# Autodesk Inventor assembly: Drive Base Assembly
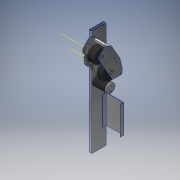
[picture p0: Inventor's stored thumbnail of the model, 180x180]
Saved by Autodesk Inventor 2019.4 (Build 234330000, 330)
## iProperties
Created: 2019-11-02
Part Number: Drive Base Assembly
Document SubType Name: Assembly
Designer: admin
Author: admin
## Documents named in this file (13)
- C:\Users\admin\Desktop\FRC 2020 Engineering\GitHub\7738-CAD-prep\Butterfly Drive Mk2\Butterfly Base\Drive Base Assembly.iam
- C:\Users\admin\Desktop\FRC 2020 Engineering\GitHub\7738-CAD-prep\Butterfly Drive Mk2\Butterfly Base\Main Axle.ipt
- C:\Users\admin\Desktop\FRC 2020 Engineering\GitHub\7738-CAD-prep\Butterfly Drive Mk2\Butterfly Module\Butterfly Drive Module.iam
- C:\Users\admin\Desktop\FRC 2020 Engineering\GitHub\7738-CAD-prep\Butterfly Drive Mk2\Butterfly Base\Side Extrusion.ipt
- C:\Users\admin\Desktop\FRC 2020 Engineering\GitHub\7738-CAD-prep\Butterfly Drive Mk2\Butterfly Base\am-0255 2.5inch CIM Motor.ipt
- C:\Users\admin\Desktop\FRC 2020 Engineering\GitHub\7738-CAD-prep\Butterfly Drive Mk2\Butterfly Base\Mottor Protection Piece.ipt
- C:\Users\admin\Desktop\FRC 2020 Engineering\GitHub\7738-CAD-prep\Butterfly Drive Mk2\Butterfly Base\Drive Base Assembly\Design Accelerator\Spur Gears1.iam
- C:\Users\admin\Desktop\FRC 2020 Engineering\GitHub\7738-CAD-prep\Butterfly Drive Mk2\Butterfly Base\Drive Base Assembly\Design Accelerator\Spur Gears2.iam
- C:\Users\admin\Desktop\FRC 2020 Engineering\GitHub\7738-CAD-prep\Butterfly Drive Mk2\Butterfly Base\Drive Base Assembly\Design Accelerator\Spur Gears3.iam
- C:\Users\admin\Desktop\FRC 2020 Engineering\GitHub\7738-CAD-prep\Butterfly Drive Mk2\Butterfly Base\F6004.ipt
- C:\Users\admin\Desktop\FRC 2020 Engineering\GitHub\7738-CAD-prep\Butterfly Drive Mk2\Butterfly Base\F6802.ipt
- C:\Users\admin\Desktop\FRC 2020 Engineering\GitHub\7738-CAD-prep\Butterfly Drive Mk2\Butterfly Base\F6800Z 10mm ID Flange.ipt
- C:\Users\admin\Desktop\FRC 2020 Engineering\GitHub\7738-CAD-prep\Butterfly Drive Mk2\Butterfly Base\Gear Protection Piece.ipt
## Components (12 placed, 10 different names)
1. Main Axle:1 — Mate:1, Flush:1, Mate:24, Mate:28, Mate:29, Mate:30
2. Butterfly Drive Module:1 [sub-assembly] — Mate:1, Flush:1, Mate:2, Angle:1, Mate:7
3. Side Extrusion:1 — Mate:2, Mate:5, Flush:2, Angle:1, Mate:8, Mate:10, Flush:3, Flush:4, Mate:17, Mate:19, Angle:2, Mate:23, Mate:27, Mate:31, Mate:32
4. am-0255 2.5inch CIM Motor:1 — Mate:12, Mate:17, Mate:19
5. Mottor Protection Piece:1 — Mate:5, Flush:2
6. Spur Gears:1 [sub-assembly] — Mate:11, Mate:14, Mate:16, Mate:18, Mate:20, Mate:21
7. Spur Gears:2 [sub-assembly] — Mate:7, Mate:8, Mate:11, Mate:18
8. Spur Gears:3 [sub-assembly] — Mate:12, Mate:14, Mate:16
9. F6004:1 — Mate:23, Mate:24, Mate:27
10. F6802:1 — Mate:33, Mate:34
11. F6800Z 10mm ID Flange:1 — Mate:28, Mate:29
12. Gear Protection Piece:1 — Mate:30, Mate:31, Mate:32, Mate:33, Mate:34
## Relationships (31: Mate 25, Flush 4, Angle 2)
- Mate:1: Main Axle:1 ↔ Butterfly Drive Module:1
- Flush:1: Main Axle:1 ↔ Butterfly Drive Module:1
- Mate:2 (6.5 mm): Butterfly Drive Module:1 ↔ Side Extrusion:1
- Mate:5 (0.5 mm): Side Extrusion:1 ↔ Mottor Protection Piece:1
- Flush:2: Side Extrusion:1 ↔ Mottor Protection Piece:1
- Angle:1 (30 deg): Butterfly Drive Module:1 ↔ Side Extrusion:1
- Mate:7: Butterfly Drive Module:1 ↔ Spur Gears:2
- Mate:8 (7 mm): Side Extrusion:1 ↔ Spur Gears:2
- Mate:10: Side Extrusion:1
- Flush:3: Side Extrusion:1
- Flush:4: Side Extrusion:1
- Mate:11 (3 mm): Spur Gears:1 ↔ Spur Gears:2
- Mate:12: am-0255 2.5inch CIM Motor:1 ↔ Spur Gears:3
- Mate:14 (3 mm): Spur Gears:1 ↔ Spur Gears:3
- Mate:16: Spur Gears:1 ↔ Spur Gears:3
- Mate:17 (0.3 mm): Side Extrusion:1 ↔ am-0255 2.5inch CIM Motor:1
- Mate:18: Spur Gears:1 ↔ Spur Gears:2
- Mate:19: Side Extrusion:1 ↔ am-0255 2.5inch CIM Motor:1
- Mate:20: Spur Gears:1
- Mate:21: Spur Gears:1
- Angle:2 (0 deg): Side Extrusion:1
- Mate:23: Side Extrusion:1 ↔ F6004:1
- Mate:24: Main Axle:1 ↔ F6004:1
- Mate:27 (0.3 mm): Side Extrusion:1 ↔ F6004:1
- Mate:28: Main Axle:1 ↔ F6800Z 10mm ID Flange:1
- Mate:29 (0.3 mm): Main Axle:1 ↔ F6800Z 10mm ID Flange:1
- Mate:30: Main Axle:1 ↔ Gear Protection Piece:1
- Mate:31 (0.2 mm): Side Extrusion:1 ↔ Gear Protection Piece:1
- Mate:32: Side Extrusion:1 ↔ Gear Protection Piece:1
- Mate:33: F6802:1 ↔ Gear Protection Piece:1
- Mate:34 (0.2 mm): F6802:1 ↔ Gear Protection Piece:1
